# Autodesk Inventor assembly: ElectronicsBoard
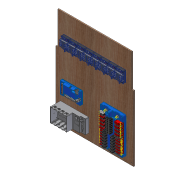
[picture p0: Inventor's stored thumbnail of the model, 180x180]
Saved by Autodesk Inventor 2012 (Build 160160000, 160)
## iProperties
Created: 2012-11-22
Part Number: ElectronicsBoard
Document SubType Name: Assembly
Designer: JesseK
Author: JesseK
## Documents named in this file (6)
- Z:\UserData\Documents\Inventor\team1885frc\Robot2013\DriveTrainProto\ElectronicsBoard.iam
- Z:\UserData\Documents\Inventor\team1885frc\Robot2013\DriveTrainProto\ElectronicsBoard.ipt
- Z:\UserData\Documents\Inventor\team1885frc\AndyMark\Talon.ipt
- Z:\UserData\Documents\Inventor\team1885frc\Electronics\cRIO_4Slot\Imported Components\cu_crio-9075_4-slot\cu_crio-9075_4-slot.ipt
- Z:\UserData\Documents\Inventor\team1885frc\Electronics\PowerDistributionBoard\elc_Power_Distro_inv.iam
- Z:\UserData\Documents\Inventor\team1885frc\Electronics\DigitalSidecar\elc_Digital_Sidecar_inv.iam
## Components (12 placed, 5 different names)
1. ElectronicsBoard:1 — Mate:1, Mate:2, Mate:3, Mate:4, Mate:6, Mate:7, Mate:9, Mate:10, Mate:18, Mate:19, Mate:20, Flush:10, Flush:11
2. Talon:1 — Mate:3, Flush:5, Flush:6, Mate:15, Flush:7, Mate:16
3. Talon:2 — Mate:7, Flush:4, Mate:12, Mate:13
4. Talon:3 — Mate:4, Flush:2, Mate:11
5. Talon:5 — Mate:10, Flush:6, Mate:14, Mate:15
6. Talon:6 — Mate:9, Flush:3, Flush:4, Flush:5, Mate:13, Mate:14
7. Talon:7 — Mate:1, Flush:7, Flush:8, Mate:16, Mate:17
8. Talon:8 — Mate:2, Flush:2, Flush:3, Mate:11, Mate:12
9. Talon:9 — Mate:6, Flush:8, Mate:17
10. cu_crio-9075_4-slot:1 — Mate:18, Flush:11
11. elc_Power_Distro_inv:1 [sub-assembly] — Mate:19
12. elc_Digital_Sidecar_inv:1 [sub-assembly] — Mate:20, Flush:10
## Relationships (27: Mate 18, Flush 9)
- Mate:1: ElectronicsBoard:1 ↔ Talon:7
- Mate:2: ElectronicsBoard:1 ↔ Talon:8
- Mate:3: ElectronicsBoard:1 ↔ Talon:1
- Mate:4: ElectronicsBoard:1 ↔ Talon:3
- Mate:6: ElectronicsBoard:1 ↔ Talon:9
- Mate:7: ElectronicsBoard:1 ↔ Talon:2
- Mate:9: ElectronicsBoard:1 ↔ Talon:6
- Mate:10: ElectronicsBoard:1 ↔ Talon:5
- Flush:2: Talon:3 ↔ Talon:8
- Flush:3: Talon:6 ↔ Talon:8
- Flush:4: Talon:2 ↔ Talon:6
- Flush:5: Talon:1 ↔ Talon:6
- Flush:6: Talon:1 ↔ Talon:5
- Mate:11: Talon:3 ↔ Talon:8
- Mate:12: Talon:2 ↔ Talon:8
- Mate:13: Talon:2 ↔ Talon:6
- Mate:14: Talon:5 ↔ Talon:6
- Mate:15: Talon:1 ↔ Talon:5
- Flush:7: Talon:1 ↔ Talon:7
- Flush:8: Talon:7 ↔ Talon:9
- Mate:16: Talon:1 ↔ Talon:7
- Mate:17: Talon:7 ↔ Talon:9
- Mate:18: ElectronicsBoard:1 ↔ cu_crio-9075_4-slot:1
- Mate:19: ElectronicsBoard:1 ↔ elc_Power_Distro_inv:1
- Mate:20: ElectronicsBoard:1 ↔ elc_Digital_Sidecar_inv:1
- Flush:10 (50.8 mm): ElectronicsBoard:1 ↔ elc_Digital_Sidecar_inv:1
- Flush:11 (101.6 mm): ElectronicsBoard:1 ↔ cu_crio-9075_4-slot:1
